# Autodesk Inventor assembly: 霍爾
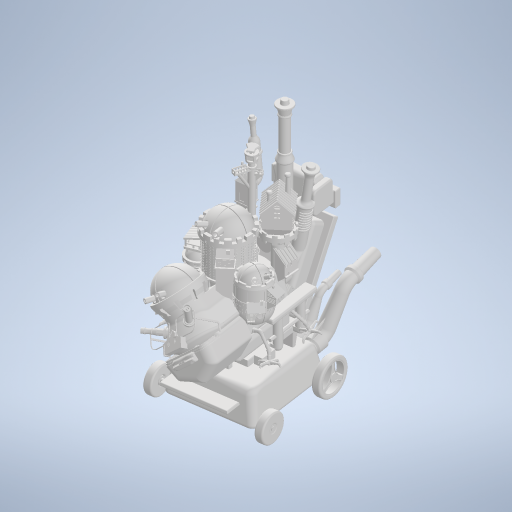
[picture p0: Inventor's stored thumbnail of the model, 512x512]
Saved by Autodesk Inventor 2024 (Build 280153000, 153)
## iProperties
Created: 2024-05-18
Part Number: 霍爾
Document SubType Name: Assembly
Designer: User
Author: User
## Documents named in this file (34)
- C:\Users\User\Documents\Inventor\construction\霍爾.iam
- C:\Users\User\Documents\Inventor\construction\柱-1 磚-1.ipt
- C:\Users\User\Documents\Inventor\construction\柱-1 磚-2.ipt
- C:\Users\User\Documents\Inventor\construction\屋頂-1.ipt
- C:\Users\User\Documents\Inventor\construction\屋-1 base.ipt
- C:\Users\User\Documents\Inventor\construction\不知道取啥.ipt
- C:\Users\User\Documents\Inventor\construction\屋1 物2.ipt
- C:\Users\User\Documents\Inventor\construction\屋1 物1 柱1.ipt
- C:\Users\User\Documents\Inventor\construction\屋1 物1 base.ipt
- C:\Users\User\Documents\Inventor\construction\屋1 物3.ipt
- C:\Users\User\Documents\Inventor\construction\連接件1.ipt
- C:\Users\User\Documents\Inventor\construction\頭組.iam
- C:\Users\User\Documents\Inventor\construction\屋-2.iam
- C:\Users\User\Documents\Inventor\construction\桿子.ipt
- C:\Users\User\Documents\Inventor\construction\另屋1.ipt
- C:\Users\User\Documents\Inventor\construction\另屋1 base.ipt
- C:\Users\User\Documents\Inventor\construction\body.ipt
- C:\Users\User\Documents\Inventor\construction\下巴.ipt
- C:\Users\User\Documents\Inventor\construction\另屋1 物1.ipt
- C:\Users\User\Documents\Inventor\construction\背部建築.ipt
- C:\Users\User\Documents\Inventor\construction\背部建築 base.ipt
- C:\Users\User\Documents\Inventor\construction\背 物1.ipt
- C:\Users\User\Documents\Inventor\construction\背 物2.ipt
- C:\Users\User\Documents\Inventor\construction\塔1.ipt
- C:\Users\User\Documents\Inventor\construction\塔2.ipt
- C:\Users\User\Documents\Inventor\construction\塔3.ipt
- C:\Users\User\Documents\Inventor\construction\背屋.ipt
- C:\Users\User\Documents\Inventor\construction\眼 左.ipt
- C:\Users\User\Documents\Inventor\construction\眼 右.ipt
- C:\Users\User\Documents\Inventor\construction\眼鏡.ipt
- C:\Users\User\Documents\Inventor\construction\輪椅.ipt
- C:\Users\User\Documents\Inventor\construction\排氣管 1.ipt
- C:\Users\User\Documents\Inventor\construction\排氣管 2.ipt
- C:\Users\User\Documents\Inventor\construction\腳.ipt
## Components (66 placed, 33 different names)
1. 屋1 物1:1 — 貼合:6, 貼合:7, 齊平:1, 貼合:11, 貼合:17
2. 屋頂-1:2 — 貼合:2, 貼合:3, 貼合:25, 貼合:27
3. 屋-1 base:1 — 貼合:4, 貼合:5, 貼合:6
4. 屋1 物2:1 — 齊平:1, 貼合:10
5. 屋1 物1 柱1:1 — 貼合:11, 貼合:12, 貼合:14
6. 屋1 物1 柱1:2 — 貼合:12, 貼合:13, 貼合:14, 貼合:15
7. 屋1 物1 柱1:3 — 貼合:13, 貼合:15, 貼合:16
8. 屋1 物1 base:1 — 貼合:16, 貼合:17
9. 屋1 物3:1 — 貼合:18
10. 連接件1:1 — 貼合:24
11. 頭組:1 [sub-assembly] — 貼合:23, 貼合:29, 齊平:2, 貼合:39, 貼合:40, 貼合:41, 貼合:42, 貼合:43, 齊平:3
12. 屋-2:1 [sub-assembly] — 貼合:22
13. 桿子:1 — 貼合:25
14. 另屋1:1 — 貼合:26, 貼合:27, 貼合:28
15. 另屋1 base:1 — 貼合:28
16. body:1 — 貼合:29, 貼合:30, 貼合:31, 貼合:37, 貼合:38, 貼合:44, 齊平:4, 貼合:49, 貼合:50, 貼合:51, 貼合:52
17. 下巴:1 — 齊平:2, 貼合:30
18. 另屋1 物1:1
19. 背部建築:1 — 貼合:31, 貼合:32, 貼合:33, 貼合:34, 貼合:35, 貼合:36
20. 背部建築 base:1 — 貼合:32
21. 背 物1:1 — 貼合:33
22. 背 物2:1 — 貼合:34
23. 塔1:1 — 貼合:35
24. 塔2:1 — 貼合:36
25. 塔3:1 — 貼合:37
26. 背屋:1 — 貼合:38
27. 眼 左:1 — 貼合:39, 貼合:40
28. 眼 右:1 — 貼合:41, 貼合:42
29. 眼鏡:1 — 貼合:43, 齊平:3
30. 輪椅:1 — 貼合:44, 齊平:4, 貼合:45, 貼合:46, 貼合:47, 貼合:48
31. 排氣管 1:1 — 貼合:45
32. 排氣管 1:2 — 貼合:46
33. 排氣管 2:1 — 貼合:47
34. 排氣管 2:2 — 貼合:48
35. 腳:1 — 貼合:49
36. 腳:2 — 貼合:50
37. 腳:3 — 貼合:51
38. 腳:4 — 貼合:52
39. 柱-1 磚-1:1 — 貼合:1, 貼合:4, 貼合:5
40. 柱-1 磚-2:1 — 貼合:1
41. 柱-1 磚-1:3
42. 柱-1 磚-2:3
43. 柱-1 磚-1:4
44. 柱-1 磚-2:4
45. 柱-1 磚-1:5
46. 柱-1 磚-2:5
47. 柱-1 磚-1:6
48. 柱-1 磚-2:6 — 貼合:7
49. 柱-1 磚-1:7
50. 柱-1 磚-2:7
51. 柱-1 磚-1:8 — 貼合:24
52. 柱-1 磚-2:8
53. 柱-1 磚-1:9
54. 柱-1 磚-2:9
55. 柱-1 磚-1:10 — 貼合:18, 貼合:22
56. 柱-1 磚-2:10 — 貼合:23
57. 柱-1 磚-1:11 — 貼合:10
58. 柱-1 磚-2:11
59. 柱-1 磚-1:12 — 貼合:26
60. 柱-1 磚-2:12
61. 柱-1 磚-1:13
62. 柱-1 磚-2:13
63. 柱-1 磚-1:14
64. 柱-1 磚-2:14
65. 柱-1 磚-1:15
66. 柱-1 磚-2:15 — 貼合:2, 貼合:3
## Component patterns: (14 elements, first: 柱-1 磚-1:1 + 柱-1 磚-2:1)
## Relationships (51: Mate 47, Flush 4)
- 貼合:1 [Mate]: 柱-1 磚-1:1 ↔ 柱-1 磚-2:1
- 貼合:2 [Mate]: 屋頂-1:2 ↔ 柱-1 磚-2:15
- 貼合:3 [Mate]: 屋頂-1:2 ↔ 柱-1 磚-2:15
- 貼合:4 [Mate]: 屋-1 base:1 ↔ 柱-1 磚-1:1
- 貼合:5 [Mate]: 屋-1 base:1 ↔ 柱-1 磚-1:1
- 貼合:6 [Mate]: 屋1 物1:1 ↔ 屋-1 base:1
- 貼合:7 [Mate] (-55 mm): 屋1 物1:1 ↔ 柱-1 磚-2:6
- 齊平:1 [Flush] (5 mm): 屋1 物1:1 ↔ 屋1 物2:1
- 貼合:10 [Mate] (-54 mm): 屋1 物2:1 ↔ 柱-1 磚-1:11
- 貼合:11 [Mate]: 屋1 物1:1 ↔ 屋1 物1 柱1:1
- 貼合:12 [Mate]: 屋1 物1 柱1:1 ↔ 屋1 物1 柱1:2
- 貼合:13 [Mate]: 屋1 物1 柱1:2 ↔ 屋1 物1 柱1:3
- 貼合:14 [Mate]: 屋1 物1 柱1:1 ↔ 屋1 物1 柱1:2
- 貼合:15 [Mate]: 屋1 物1 柱1:2 ↔ 屋1 物1 柱1:3
- 貼合:16 [Mate]: 屋1 物1 柱1:3 ↔ 屋1 物1 base:1
- 貼合:17 [Mate]: 屋1 物1:1 ↔ 屋1 物1 base:1
- 貼合:18 [Mate]: 屋1 物3:1 ↔ 柱-1 磚-1:10
- 貼合:22 [Mate]: 屋-2:1 ↔ 柱-1 磚-1:10
- 貼合:23 [Mate] (6 mm): 頭組:1 ↔ 柱-1 磚-2:10
- 貼合:24 [Mate] (-5 mm): 連接件1:1 ↔ 柱-1 磚-1:8
- 貼合:25 [Mate] (-100 mm): 屋頂-1:2 ↔ 桿子:1
- 貼合:26 [Mate] (5 mm): 另屋1:1 ↔ 柱-1 磚-1:12
- 貼合:27 [Mate] (-18 mm): 屋頂-1:2 ↔ 另屋1:1
- 貼合:28 [Mate]: 另屋1:1 ↔ 另屋1 base:1
- 貼合:29 [Mate]: 頭組:1 ↔ body:1
- 齊平:2 [Flush] (40 mm): 頭組:1 ↔ 下巴:1
- 貼合:30 [Mate]: body:1 ↔ 下巴:1
- 貼合:31 [Mate]: body:1 ↔ 背部建築:1
- 貼合:32 [Mate]: 背部建築:1 ↔ 背部建築 base:1
- 貼合:33 [Mate]: 背部建築:1 ↔ 背 物1:1
- 貼合:34 [Mate]: 背部建築:1 ↔ 背 物2:1
- 貼合:35 [Mate]: 背部建築:1 ↔ 塔1:1
- 貼合:36 [Mate]: 背部建築:1 ↔ 塔2:1
- 貼合:37 [Mate]: body:1 ↔ 塔3:1
- 貼合:38 [Mate]: body:1 ↔ 背屋:1
- 貼合:39 [Mate]: 頭組:1 ↔ 眼 左:1
- 貼合:40 [Mate]: 頭組:1 ↔ 眼 左:1
- 貼合:41 [Mate]: 頭組:1 ↔ 眼 右:1
- 貼合:42 [Mate]: 頭組:1 ↔ 眼 右:1
- 貼合:43 [Mate] (-2 mm): 頭組:1 ↔ 眼鏡:1
- 齊平:3 [Flush] (20 mm): 頭組:1 ↔ 眼鏡:1
- 貼合:44 [Mate]: body:1 ↔ 輪椅:1
- 齊平:4 [Flush]: body:1 ↔ 輪椅:1
- 貼合:45 [Mate]: 輪椅:1 ↔ 排氣管 1:1
- 貼合:46 [Mate]: 輪椅:1 ↔ 排氣管 1:2
- 貼合:47 [Mate]: 輪椅:1 ↔ 排氣管 2:1
- 貼合:48 [Mate]: 輪椅:1 ↔ 排氣管 2:2
- 貼合:49 [Mate]: body:1 ↔ 腳:1
- 貼合:50 [Mate]: body:1 ↔ 腳:2
- 貼合:51 [Mate]: body:1 ↔ 腳:3
- 貼合:52 [Mate]: body:1 ↔ 腳:4
